# Autodesk Inventor assembly: platform
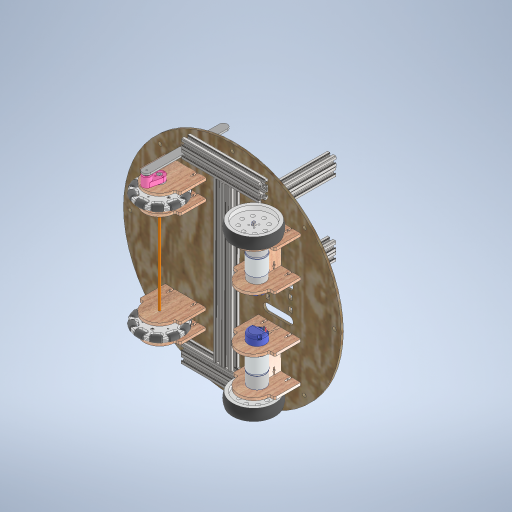
[picture p0: Inventor's stored thumbnail of the model, 512x512]
Saved by Autodesk Inventor 2023.1 (Build 271208000, 208)
## iProperties
Created: 2023-03-13
Part Number: platform
Document SubType Name: Assembly
Designer: User
Author: User
## Documents named in this file (22)
- C:\Users\DELL\Desktop\Cheburashka_construction\Cheburashka\cheb\platform.iam
- C:\Users\DELL\Desktop\Cheburashka_construction\Cheburashka\cheb\Osn. platform.ipt
- C:\Users\DELL\Desktop\Cheburashka_construction\Cheburashka\cheb\motor1.ipt
- C:\Users\DELL\Desktop\Cheburashka_construction\Cheburashka\cheb\motor2.ipt
- C:\Users\DELL\Desktop\Cheburashka_construction\Cheburashka\cheb\motor3.ipt
- C:\Users\DELL\Desktop\Cheburashka_construction\Cheburashka\cheb\wheel1.ipt
- C:\Users\DELL\Desktop\Cheburashka_construction\Cheburashka\cheb\Импорт\44260_txm torquenado dc motor_MIR2.ipt
- C:\Users\DELL\Desktop\Cheburashka_construction\Cheburashka\cheb\Импорт\36466_txm-4 inch omni wheel.ipt
- C:\Users\DELL\Desktop\Cheburashka_construction\Cheburashka\cheb\Импорт\39055_txm-4 inch wheel_MIR1.ipt
- C:\Users\DELL\Desktop\Cheburashka_construction\Cheburashka\cheb\motor1_MIR3.ipt
- C:\Users\DELL\Desktop\Cheburashka_construction\Cheburashka\cheb\motor2_MIR3.ipt
- C:\Users\DELL\Desktop\Cheburashka_construction\Cheburashka\cheb\motor3_MIR3.ipt
- C:\Users\DELL\Desktop\Cheburashka_construction\Cheburashka\cheb\Импорт\44260_txm torquenado dc motor_MIR2_MIR.ipt
- C:\Users\DELL\Desktop\Cheburashka_construction\Cheburashka\cheb\wheel1_MIR.ipt
- C:\Users\DELL\Desktop\Cheburashka_construction\Cheburashka\cheb\Импорт\36466_txm-4 inch omni wheel_MIR2.ipt
- C:\Users\DELL\Desktop\Cheburashka_construction\Cheburashka\cheb\Импорт\39055_txm-4 inch wheel_MIR1_MIR.ipt
- C:\Users\DELL\Desktop\Cheburashka_construction\Cheburashka\cheb\Импорт\224HX-Konstruktsionnyy-profil-20kh20H.iam
- C:\Users\DELL\Desktop\Cheburashka_construction\Cheburashka\cheb\кривошип.ipt
- C:\Users\DELL\Desktop\Cheburashka_construction\Cheburashka\cheb\ось колес2.ipt
- C:\Users\DELL\Desktop\Cheburashka_construction\Cheburashka\cheb\akfytw2.ipt
- C:\Users\DELL\Desktop\Cheburashka_construction\Cheburashka\cheb\подшипник2.ipt
- C:\Users\DELL\Desktop\Cheburashka_construction\Cheburashka\cheb\шатун22.ipt
## Components (28 placed, 21 different names)
1. Osn. platform:1 — Совмещение:1, Совмещение:2, Совмещение:5, Совмещение:8, Совмещение:13, Совмещение:17, Совмещение:29, Совмещение:30, Совмещение:31, Совмещение:32, Совмещение:33, Совмещение:34, Совмещение:35, Совмещение:36, Совмещение:37, Совмещение:38, Заподлицо:2, Совмещение:45, Совмещение:46, Заподлицо:3, Совмещение:47, Совмещение:48, Совмещение:49, Совмещение:50, Совмещение:51, Совмещение:53
2. motor1:1 — Совмещение:2, Совмещение:31, Совмещение:32
3. motor2:1 — Совмещение:5, Совмещение:29, Совмещение:30
4. motor3:1 — Совмещение:8, Совмещение:11, Совмещение:12, Совмещение:22, Совмещение:33, Совмещение:34
5. 44260_txm torquenado dc motor_MIR2:1 — Совмещение:11, Совмещение:12, Совмещение:21
6. wheel1:1 — Совмещение:13, Совмещение:19, Совмещение:37, Совмещение:38, Совмещение:88
7. wheel1:2 — Совмещение:17, Совмещение:35, Совмещение:36
8. 36466_txm-4 inch omni wheel:1 — Совмещение:19
9. 39055_txm-4 inch wheel_MIR1:1 — Совмещение:21, Совмещение:22
10. motor1_MIR3:1
11. motor2_MIR3:1
12. motor3_MIR3:1 — Совмещение:23, Совмещение:24, Совмещение:27
13. 44260_txm torquenado dc motor_MIR2_MIR:1 — Совмещение:23, Совмещение:24, Совмещение:28
14. wheel1_MIR:1 — Совмещение:25, Совмещение:26, Заподлицо:24
15. wheel1_MIR:2 — Совмещение:87
16. 36466_txm-4 inch omni wheel_MIR2:1 — Совмещение:25, Совмещение:26
17. 39055_txm-4 inch wheel_MIR1_MIR:1 — Совмещение:27, Совмещение:28
18. 224HX-Konstruktsionnyy-profil-20kh20H:1 [sub-assembly] — Заподлицо:2, Совмещение:45, Совмещение:46
19. 224HX-Konstruktsionnyy-profil-20kh20H:3 [sub-assembly] — Совмещение:49, Совмещение:50, Совмещение:52, Совмещение:54
20. 224HX-Konstruktsionnyy-profil-20kh20H:4 [sub-assembly] — Заподлицо:3, Совмещение:47, Совмещение:48
21. 224HX-Konstruktsionnyy-profil-20kh20H:5 [sub-assembly] — Совмещение:51, Совмещение:52
22. 224HX-Konstruktsionnyy-profil-20kh20H:6 [sub-assembly] — Совмещение:53, Совмещение:54
23. кривошип:1 — Совмещение:90, Совмещение:91, Совмещение:92, Совмещение:93, Совмещение:96
24. ось колес2:1 — Совмещение:87, Заподлицо:24, Совмещение:89
25. akfytw2:1 — Совмещение:88, Совмещение:89, Совмещение:90, Совмещение:91
26. подшипник2:1 — Совмещение:92, Совмещение:93, Совмещение:94
27. подшипник2:2 — Совмещение:94, Совмещение:95
28. шатун22:1 — Совмещение:95, Совмещение:96
## Relationships (50: Mate 47, Flush 3)
- Совмещение:1 [Mate]: Osn. platform:1
- Совмещение:2 [Mate]: Osn. platform:1 ↔ motor1:1
- Совмещение:5 [Mate]: Osn. platform:1 ↔ motor2:1
- Совмещение:8 [Mate]: Osn. platform:1 ↔ motor3:1
- Совмещение:11 [Mate]: motor3:1 ↔ 44260_txm torquenado dc motor_MIR2:1
- Совмещение:12 [Mate]: motor3:1 ↔ 44260_txm torquenado dc motor_MIR2:1
- Совмещение:13 [Mate]: Osn. platform:1 ↔ wheel1:1
- Совмещение:17 [Mate]: Osn. platform:1 ↔ wheel1:2
- Совмещение:19 [Mate]: wheel1:1 ↔ 36466_txm-4 inch omni wheel:1
- Совмещение:21 [Mate]: 44260_txm torquenado dc motor_MIR2:1 ↔ 39055_txm-4 inch wheel_MIR1:1
- Совмещение:22 [Mate] (15 mm): motor3:1 ↔ 39055_txm-4 inch wheel_MIR1:1
- Совмещение:23 [Mate]: motor3_MIR3:1 ↔ 44260_txm torquenado dc motor_MIR2_MIR:1
- Совмещение:24 [Mate]: motor3_MIR3:1 ↔ 44260_txm torquenado dc motor_MIR2_MIR:1
- Совмещение:25 [Mate] (10 mm): wheel1_MIR:1 ↔ 36466_txm-4 inch omni wheel_MIR2:1
- Совмещение:26 [Mate]: wheel1_MIR:1 ↔ 36466_txm-4 inch omni wheel_MIR2:1
- Совмещение:27 [Mate] (15 mm): motor3_MIR3:1 ↔ 39055_txm-4 inch wheel_MIR1_MIR:1
- Совмещение:28 [Mate]: 44260_txm torquenado dc motor_MIR2_MIR:1 ↔ 39055_txm-4 inch wheel_MIR1_MIR:1
- Совмещение:29 [Mate]: Osn. platform:1 ↔ motor2:1
- Совмещение:30 [Mate]: Osn. platform:1 ↔ motor2:1
- Совмещение:31 [Mate]: Osn. platform:1 ↔ motor1:1
- Совмещение:32 [Mate]: Osn. platform:1 ↔ motor1:1
- Совмещение:33 [Mate]: Osn. platform:1 ↔ motor3:1
- Совмещение:34 [Mate]: Osn. platform:1 ↔ motor3:1
- Совмещение:35 [Mate]: Osn. platform:1 ↔ wheel1:2
- Совмещение:36 [Mate]: Osn. platform:1 ↔ wheel1:2
- Совмещение:37 [Mate]: Osn. platform:1 ↔ wheel1:1
- Совмещение:38 [Mate]: Osn. platform:1 ↔ wheel1:1
- Заподлицо:2 [Flush]: Osn. platform:1 ↔ 224HX-Konstruktsionnyy-profil-20kh20H:1
- Совмещение:45 [Mate]: Osn. platform:1 ↔ 224HX-Konstruktsionnyy-profil-20kh20H:1
- Совмещение:46 [Mate]: Osn. platform:1 ↔ 224HX-Konstruktsionnyy-profil-20kh20H:1
- Заподлицо:3 [Flush]: Osn. platform:1 ↔ 224HX-Konstruktsionnyy-profil-20kh20H:4
- Совмещение:47 [Mate]: Osn. platform:1 ↔ 224HX-Konstruktsionnyy-profil-20kh20H:4
- Совмещение:48 [Mate]: Osn. platform:1 ↔ 224HX-Konstruktsionnyy-profil-20kh20H:4
- Совмещение:49 [Mate]: Osn. platform:1 ↔ 224HX-Konstruktsionnyy-profil-20kh20H:3
- Совмещение:50 [Mate]: Osn. platform:1 ↔ 224HX-Konstruktsionnyy-profil-20kh20H:3
- Совмещение:51 [Mate]: Osn. platform:1 ↔ 224HX-Konstruktsionnyy-profil-20kh20H:5
- Совмещение:52 [Mate]: 224HX-Konstruktsionnyy-profil-20kh20H:3 ↔ 224HX-Konstruktsionnyy-profil-20kh20H:5
- Совмещение:53 [Mate]: Osn. platform:1 ↔ 224HX-Konstruktsionnyy-profil-20kh20H:6
- Совмещение:54 [Mate]: 224HX-Konstruktsionnyy-profil-20kh20H:3 ↔ 224HX-Konstruktsionnyy-profil-20kh20H:6
- Совмещение:87 [Mate]: wheel1_MIR:2 ↔ ось колес2:1
- Заподлицо:24 [Flush]: wheel1_MIR:1 ↔ ось колес2:1
- Совмещение:88 [Mate]: wheel1:1 ↔ akfytw2:1
- Совмещение:89 [Mate]: ось колес2:1 ↔ akfytw2:1
- Совмещение:90 [Mate]: кривошип:1 ↔ akfytw2:1
- Совмещение:91 [Mate]: кривошип:1 ↔ akfytw2:1
- Совмещение:92 [Mate]: кривошип:1 ↔ подшипник2:1
- Совмещение:93 [Mate]: кривошип:1 ↔ подшипник2:1
- Совмещение:94 [Mate]: подшипник2:1 ↔ подшипник2:2
- Совмещение:95 [Mate]: подшипник2:2 ↔ шатун22:1
- Совмещение:96 [Mate] (4 mm): кривошип:1 ↔ шатун22:1
